# Autodesk Inventor assembly: M2-脚ギア1段目
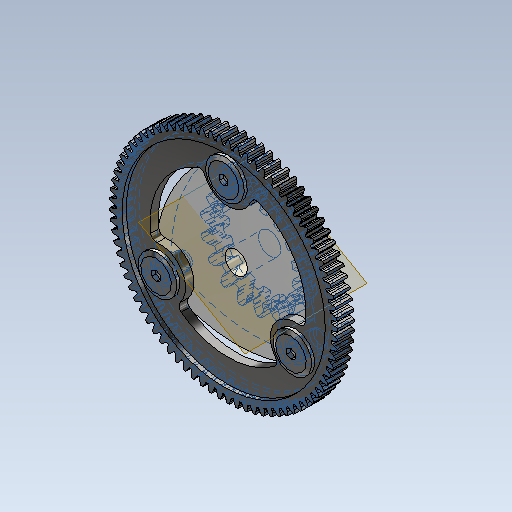
[picture p0: Inventor's stored thumbnail of the model, 512x512]
Saved by Autodesk Inventor 2020 (Build 240168000, 168)
## iProperties
Created: 2020-10-28
Part Number: M2-脚ギア1段目
Document SubType Name: Assembly
Designer: AA19065
Mass: 18.795 g
Surface Area: 48.4895 cm^2
Volume: 3.93772 cm^3
Density: 4.77307 g/cm^3
Author: AA19065
## Documents named in this file (4)
- C:\Users\happy\OneDrive\ドキュメント\賢一ファイル\SRDC\試作10-2\アセンブリ\M2-脚ギア1段目.iam
- C:\Users\happy\OneDrive\ドキュメント\賢一ファイル\SRDC\試作10-2\ギア\M2-m1z17.ipt
- C:\Users\happy\OneDrive\ドキュメント\賢一ファイル\SRDC\試作10-2\ギア\M2-歯車m0.5,z80.ipt
- C:\Users\happy\OneDrive\ドキュメント\賢一ファイル\SRDC\試作10-2\ねじ\M2-M3L4　超極低頭.ipt
## Components (5 placed, 3 different names)
1. M2-m1z17:1 — 挿入:2, 挿入:1
2. M2-歯車m0.5,z80:1 — 挿入:2, 挿入:1, 挿入:3, 挿入:4, 挿入:5
3. M2-M3L4　超極低頭:1 — 挿入:3
4. M2-M3L4　超極低頭:2 — 挿入:4
5. M2-M3L4　超極低頭:3 — 挿入:5
## Relationships (5: Insert 5)
- 挿入:2 [Insert]: M2-m1z17:1 ↔ M2-歯車m0.5,z80:1
- 挿入:1 [Insert]: M2-m1z17:1 ↔ M2-歯車m0.5,z80:1
- 挿入:3 [Insert]: M2-歯車m0.5,z80:1 ↔ M2-M3L4　超極低頭:1
- 挿入:4 [Insert]: M2-歯車m0.5,z80:1 ↔ M2-M3L4　超極低頭:2
- 挿入:5 [Insert]: M2-歯車m0.5,z80:1 ↔ M2-M3L4　超極低頭:3
